# Autodesk Inventor assembly: 90-Degree-Metal-Corner
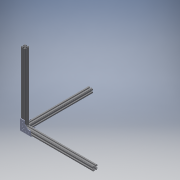
[picture p0: Inventor's stored thumbnail of the model, 180x180]
Saved by Autodesk Inventor 2017.3 (Build 213256000, 256)
## iProperties
Created: 2018-01-04
Part Number: 90-Degree-Metal-Corner
Document SubType Name: Assembly
Designer: pranav
Author: pranav
## iProperties of the stored document REV-41-1431.ipt
Created: 2017-04-10
Part Number: REV-41-1431
Material: Generic
Document SubType Name: Modeling
Designer: pranav
Density: 1 g/cm^3
Appearance: Default
Title: E:/Dropbox/REV Robotics/STEP Files/REV-41-1431.step
Sending System: Autodesk Translation Framework v5.2.0.2920
Preprocessor: ST-DEVELOPER v16.5
## iProperties of the stored document REV-41-1019.ipt
Created: 2015-08-20
Part Number: REV-41-1019
Material: Generic
Description: STEP AP214
Document SubType Name: Modeling
Designer: pranav
Density: 1 g/cm^3
Appearance: Default
Title: REV-41-1019_10mm.STEP
Revision Number: ANY
Sending System: SolidWorks 2014
Preprocessor: SwSTEP 2.0
## Documents named in this file (5)
- **C:\Users\pranav\Documents\Inventor\REV-Robot-CAD\90-Degree-Metal-Corner.iam*LocalDocs*xAqqwsfni2w3pepogRtnexsixEb*REV-41-1431.ipt
- **C:\Users\pranav\Documents\Inventor\REV-Robot-CAD\90-Degree-Metal-Corner.iam*LocalDocs*xEwiivjkf3oheuscs3k0ygyekJg*REV-41-1019.ipt
- C:\Users\pranav\Documents\Inventor\REV-Robot-CAD\90-Degree-Metal-Corner.iam
- C:\Users\pranav\Documents\Inventor\REV-Robot-CAD\REV Robotics\REV Robotics CAD\REV-41-1019.STEP
- C:\Users\pranav\Documents\Inventor\REV-Robot-CAD\REV Robotics\REV Robotics CAD\REV-41-1431.step
## Components (6 placed, 2 different names)
1. REV-41-1019:1 — Mate:3, Flush:5, Flush:6
2. REV-41-1019:2 — Mate:4, Flush:7, Flush:8
3. REV-41-1019:3 — Mate:5, Flush:9, Flush:10
4. REV-41-1431:1 — Mate:1, Flush:1, Flush:2, Flush:3, Flush:4, Mate:4, Flush:8, Mate:5, Flush:9
5. REV-41-1431:2 — Mate:1, Flush:1, Flush:2, Mate:2, Flush:5, Flush:7
6. REV-41-1431:3 — Mate:2, Flush:3, Flush:4, Mate:3, Flush:6, Flush:10
## Relationships (15: Flush 10, Mate 5)
- Mate:1: REV-41-1431:1 ↔ REV-41-1431:2
- Flush:1: REV-41-1431:1 ↔ REV-41-1431:2
- Flush:2: REV-41-1431:1 ↔ REV-41-1431:2
- Mate:2: REV-41-1431:2 ↔ REV-41-1431:3
- Flush:3: REV-41-1431:1 ↔ REV-41-1431:3
- Flush:4: REV-41-1431:1 ↔ REV-41-1431:3
- Mate:3: REV-41-1019:1 ↔ REV-41-1431:3
- Flush:5: REV-41-1019:1 ↔ REV-41-1431:2
- Flush:6: REV-41-1019:1 ↔ REV-41-1431:3
- Mate:4: REV-41-1019:2 ↔ REV-41-1431:1
- Flush:7: REV-41-1019:2 ↔ REV-41-1431:2
- Flush:8: REV-41-1019:2 ↔ REV-41-1431:1
- Mate:5: REV-41-1019:3 ↔ REV-41-1431:1
- Flush:9: REV-41-1019:3 ↔ REV-41-1431:1
- Flush:10: REV-41-1019:3 ↔ REV-41-1431:3
